# Autodesk Inventor assembly: EMU5 Robot
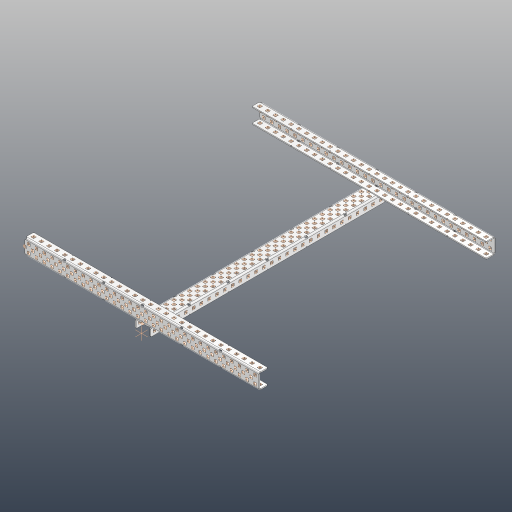
[picture p0: Inventor's stored thumbnail of the model, 512x512]
Saved by Autodesk Inventor 2023 (Build 270158000, 158)
## iProperties
Created: 2022-11-08
Part Number: EMU5 Robot
Document SubType Name: Assembly
Designer: bengo
Author: bengo
## Documents named in this file (2)
- D:\CAD Projects\emu5-15-inch-robot-cad\EMU5 Robot.iam
- D:\VEX CAD Libraries\Inventor\VEX-CAD-Inventor-1.4.0\Structure\C Channel\Aluminum 1x2x1\Alu C 1x2x1x30.ipt
## Components (3 placed, 1 different names)
1. Alu C 1x2x1x30:1 — Insert:1, Mate:1, Insert:2, Mate:2
2. Alu C 1x2x1x30:2 — Insert:1, Mate:1
3. Alu C 1x2x1x30:3 — Insert:2, Mate:2
## Relationships (4: Insert 2, Mate 2)
- Insert:1: Alu C 1x2x1x30:1 ↔ Alu C 1x2x1x30:2
- Mate:1: Alu C 1x2x1x30:1 ↔ Alu C 1x2x1x30:2
- Insert:2: Alu C 1x2x1x30:1 ↔ Alu C 1x2x1x30:3
- Mate:2: Alu C 1x2x1x30:1 ↔ Alu C 1x2x1x30:3
